# Autodesk Inventor assembly: Inner_C_Channel_26_MIR
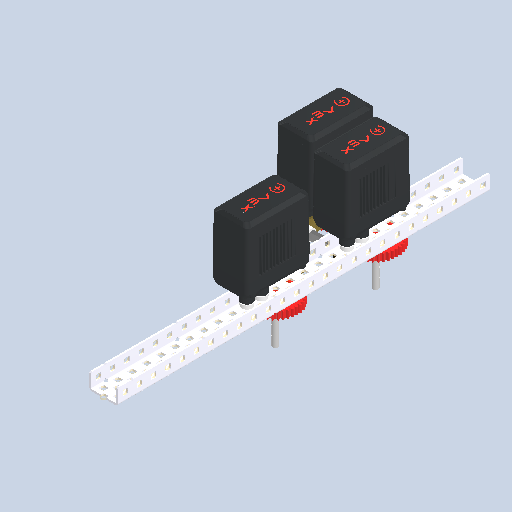
[picture p0: Inventor's stored thumbnail of the model, 512x512]
Saved by Autodesk Inventor 2025.2 (Build 292293000, 293)
## iProperties
Created: 2024-12-08
Part Number: Inner_C_Channel_26_MIR
Document SubType Name: Assembly
Designer: joshi
Author: Aditya Koduri
## Documents named in this file (9)
- C:\Users\joshi\Desktop\3388K CAD\Inner_C_Channel_26_MIR.iam
- C:\Users\joshi\Desktop\3388K CAD\VEX Main\Structure\C Channel\Aluminum 1x2x1\Alu C 1x2x1x26_MIR.ipt
- C:\Users\joshi\Desktop\3388K CAD\Motor_Section_MIR.iam
- C:\Users\joshi\Desktop\3388K CAD\VEX Main\Motion\Spacers\Spacer Nylon .313 OD\NSpacer .313 OD x .250.ipt
- C:\Users\joshi\Desktop\3388K CAD\VEX Main\Motion\Spacers\Spacer Nylon .313 OD.ipt
- C:\Users\joshi\Desktop\3388K CAD\VEX Main\Structure\Standoff\Standoff .50.ipt
- C:\Users\joshi\Desktop\3388K CAD\VEX Main\Structure\Standoff.ipt
- C:\Users\joshi\Desktop\3388K CAD\Motor_Section_Regular_Spacer_MIR.iam
- C:\Users\joshi\Desktop\3388K CAD\VEX Main\Structure\C Channel\Aluminum 1x2x1\Alu C 1x2x1x5_MIR.ipt
## Components (10 placed, 6 different names)
1. Alu C 1x2x1x26_MIR:1 — Insert:1, Insert:4, Insert:3, Insert:2, Insert:5, Insert:6
2. Motor_Section_MIR:1 [sub-assembly] — Insert:1, Insert:4
3. Motor_Section_MIR:2 [sub-assembly] — Insert:3, Insert:2
4. NSpacer .313 OD x .250:1 — Insert:7, Insert:10
5. NSpacer .313 OD x .250:2 — Insert:8, Insert:9
6. Standoff .50:1 — Insert:8, Insert:5
7. Standoff .50:2 — Insert:7, Insert:6
8. Motor_Section_Regular_Spacer_MIR:1 [sub-assembly] — Insert:12, Insert:11
9. Alu C 1x2x1x5_MIR:1 — Insert:12, Insert:11, Insert:10, Insert:9, Insert:14, Insert:13
10. Alu C 1x2x1x5_MIR:2 — Insert:14, Insert:13
## Relationships (14: Insert 14)
- Insert:1: Alu C 1x2x1x26_MIR:1 ↔ Motor_Section_MIR:1
- Insert:4: Alu C 1x2x1x26_MIR:1 ↔ Motor_Section_MIR:1
- Insert:3: Alu C 1x2x1x26_MIR:1 ↔ Motor_Section_MIR:2
- Insert:2: Alu C 1x2x1x26_MIR:1 ↔ Motor_Section_MIR:2
- Insert:8: NSpacer .313 OD x .250:2 ↔ Standoff .50:1
- Insert:5: Alu C 1x2x1x26_MIR:1 ↔ Standoff .50:1
- Insert:7: NSpacer .313 OD x .250:1 ↔ Standoff .50:2
- Insert:6: Alu C 1x2x1x26_MIR:1 ↔ Standoff .50:2
- Insert:12: Motor_Section_Regular_Spacer_MIR:1 ↔ Alu C 1x2x1x5_MIR:1
- Insert:11: Motor_Section_Regular_Spacer_MIR:1 ↔ Alu C 1x2x1x5_MIR:1
- Insert:10: NSpacer .313 OD x .250:1 ↔ Alu C 1x2x1x5_MIR:1
- Insert:9: NSpacer .313 OD x .250:2 ↔ Alu C 1x2x1x5_MIR:1
- Insert:14: Alu C 1x2x1x5_MIR:1 ↔ Alu C 1x2x1x5_MIR:2
- Insert:13: Alu C 1x2x1x5_MIR:1 ↔ Alu C 1x2x1x5_MIR:2
